# Autodesk Inventor assembly: TS_V1_Fallmagazin_gesamt
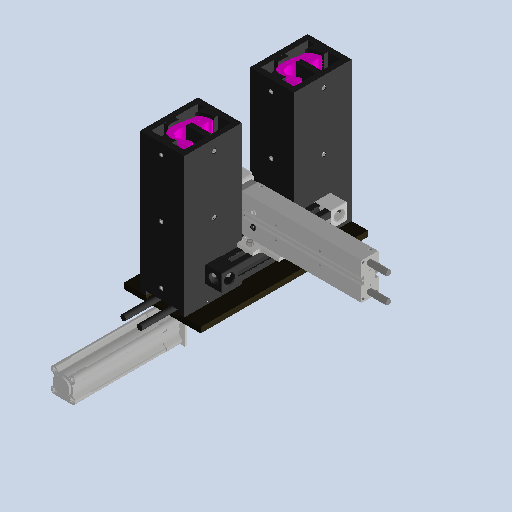
[picture p0: Inventor's stored thumbnail of the model, 512x512]
Saved by Autodesk Inventor 2025.2 (Build 292293000, 293)
## iProperties
Created: 2025-06-10
Part Number: TS_V1_Fallmagazin_gesamt
Document SubType Name: Assembly
Designer: tino
Author: tino
## Documents named in this file (30)
- C:\Users\tino\Documents_VM\Konst_CAD\CAD-Paspa\Useless Box\Eigene Bauteile\Fallmagazin\TS_V1_Fallmagazin_gesamt.iam
- C:\Users\tino\Documents_VM\Konst_CAD\CAD-Paspa\Useless Box\Eigene Bauteile\Fallmagazin\TS_V1_Fallmagazin_Boden_int.ipt
- C:\Users\tino\Documents_VM\Konst_CAD\CAD-Paspa\Useless Box\Eigene Bauteile\Fallmagazin\TS_V1_Fallmagazin_Wandung_int.ipt
- C:\Users\tino\Documents_VM\Konst_CAD\CAD-Paspa\Useless Box\Eigene Bauteile\Fallmagazin\TS_V1_Fallmagazin_Leitbleche_vorne_int.ipt
- C:\Users\tino\Documents_VM\Konst_CAD\CAD-Paspa\Useless Box\_Useless_Box\Finger.ipt
- C:\Users\tino\Documents_VM\Konst_CAD\CAD-Paspa\Useless Box\Eigene Bauteile\Fallmagazin\TS_V1_Fallmagazin_Schieber.iam
- C:\Users\tino\Documents_VM\Konst_CAD\CAD-Paspa\Useless Box\Kaufteile\Festo_Normzylinder_100\1376426 DSBC-32-100-PPVA-N3---(0).iam
- C:\Users\tino\Documents_VM\Konst_CAD\CAD-Paspa\Useless Box\Standart Bauteile\ISO 4762 - M4 x 12ISO.ipt
- C:\Users\tino\Documents_VM\Konst_CAD\CAD-Paspa\Useless Box\Standart Bauteile\ISO 4762 - M4 x 16ISO.ipt
- C:\Users\tino\Documents_VM\Konst_CAD\CAD-Paspa\Useless Box\Eigene Bauteile\Fallmagazin\TS_V1_Fallmagazin_Zylinderanbindung_int.ipt
- C:\Users\tino\Documents_VM\Konst_CAD\CAD-Paspa\Useless Box\Eigene Bauteile\Fallmagazin\TS_V1_Fallmagazin_Stopper_int.ipt
- C:\Users\tino\Documents_VM\Konst_CAD\CAD-Paspa\Useless Box\Eigene Bauteile\Fallmagazin\TS_V1_Fallmagazin_Zylinderhalter_int.ipt
- C:\Users\tino\Documents_VM\Konst_CAD\CAD-Paspa\Useless Box\Standart Bauteile\ISO 4762 - M5 x 8ISO.ipt
- C:\Users\tino\Documents_VM\Konst_CAD\CAD-Paspa\Useless Box\Standart Bauteile\ISO 4762 - M5 x 20ISO.ipt
- C:\Users\tino\Documents_VM\Konst_CAD\CAD-Paspa\Useless Box\Standart Bauteile\DIN EN ISO 2338 - 4 m6 x 10.ipt
- C:\Users\tino\Documents_VM\Konst_CAD\CAD-Paspa\Useless Box\Standart Bauteile\DIN 7991 - M5x12.ipt
- C:\Users\tino\Documents_VM\Konst_CAD\CAD-Paspa\Useless Box\Eigene Bauteile\Fallmagazin\TS_V1_Fallmagazin_Schieberanbindung_int.ipt
- C:\Users\tino\Documents_VM\Konst_CAD\CAD-Paspa\Useless Box\Eigene Bauteile\Fallmagazin\TS_V1_Fallmagazin_Verbindungsstange_int.ipt
- C:\Users\tino\Documents_VM\Konst_CAD\CAD-Paspa\Useless Box\Kaufteile\Festo_Fuehrungszylinder150_DFM_16\529120 DFM-16-150-B-P-A-KF---(0).iam
- C:\Users\tino\Documents_VM\Konst_CAD\CAD-Paspa\Useless Box\Kaufteile\DHRS-32-A - Kopie\AIS2024\1310164 DHRS-32-A---(0).iam
- C:\Users\tino\Documents_VM\Konst_CAD\CAD-Paspa\Useless Box\Eigene Bauteile\TS_Adapter_Greifer_int.ipt
- C:\Users\tino\Documents_VM\Konst_CAD\CAD-Paspa\Useless Box\Standart Bauteile\ISO 4762 - M4 x 10ISO.ipt
- C:\Users\tino\Documents_VM\Konst_CAD\CAD-Paspa\Useless Box\Eigene Bauteile\TS_Halterung_Fuehrungszylinder_int.ipt
- C:\Users\tino\Documents_VM\Konst_CAD\CAD-Paspa\Useless Box\Kaufteile\Rexroth_Profil+Winkel_30x30\Rexroth_30x30_Wuerfel\Rexroth_30x30_Wuerfel\Rexroth_30x30_Wuerfel.ipt
- C:\Users\tino\Documents_VM\Konst_CAD\CAD-Paspa\Useless Box\Kaufteile\Rexroth_Profil+Winkel_30x30\Rexroth_30x30_200_ext\Rexroth_30x30_200_ext\Rexroth_30x30_200_ext.ipt
- C:\Users\tino\Documents_VM\Konst_CAD\CAD-Paspa\Useless Box\Standart Bauteile\DIN 7991 - M8x16.ipt
- C:\Users\tino\Documents_VM\Konst_CAD\CAD-Paspa\Useless Box\Standart Bauteile\DIN 934 - M5 x 0,8.ipt
- C:\Users\tino\Documents_VM\Konst_CAD\CAD-Paspa\Useless Box\Standart Bauteile\ISO 4762 - M6 x 12ISO.ipt
- C:\Users\tino\Documents_VM\Konst_CAD\CAD-Paspa\Useless Box\Kaufteile\Rexroth_Hammermuttern\Rexroth_Hammermutter_8_M6\Rexroth_Hammermutter_8_M6\Rexroth_Hammermutter_8_M6.ipt
- C:\Users\tino\Documents_VM\Konst_CAD\CAD-Paspa\Useless Box\Standart Bauteile\DIN 913 - M5 x 6.ipt
## Components (190 placed, 29 different names)
1. TS_V1_Fallmagazin_Boden_int:1 — Passend:16, Passend:17, Passend:21, Passend:23, Passend:25, Passend:26, Passend:30, Passend:43, Passend:44, Passend:45, Passend:46, Fluchtend:18, Passend:84, Passend:85, Passend:86, Passend:87, Passend:94, Passend:96, Passend:97, Fluchtend:19, Fluchtend:20, Passend:121
2. TS_V1_Fallmagazin_Wandung_int:2 — Passend:7, Passend:8, Fluchtend:4, Winkel:1, Winkel:2, Passend:16, Passend:17, Passend:35, Passend:36, Passend:37, Passend:38, Passend:39, Passend:40, Passend:41, Passend:42, Winkel:3, Passend:130
3. TS_V1_Fallmagazin_Leitbleche_vorne_int:1 — Passend:7, Passend:8, Fluchtend:4, Tangential:2, Tangential:5, Fluchtend:12
4. TS_V1_Fallmagazin_Schieber:1 [sub-assembly] — Passend:21, Passend:25, Passend:26, Passend:53, Passend:61, Passend:62, Passend:63, Passend:64, Passend:106, Tangential:6
5. TS_V1_Fallmagazin_Schieber:2 [sub-assembly] — Passend:23, Passend:30, Passend:65, Passend:66, Passend:67, Passend:101, Passend:103, Passend:107
6. 1376426 DSBC-32-100-PPVA-N3---(0):1 [sub-assembly] — Fluchtend:18, Passend:68, Passend:69, Passend:92, Passend:93, Passend:99
7. TS_V1_Fallmagazin_Wandung_int:3 — Passend:45, Passend:46, Passend:47, Fluchtend:14, Passend:48, Passend:132, Passend:137, Passend:138
8. TS_V1_Fallmagazin_Leitbleche_vorne_int:2 — Passend:47, Fluchtend:14, Passend:48
9. TS_V1_Fallmagazin_Zylinderanbindung_int:1 — Passend:53, Passend:99, Winkel:4, Passend:104, Passend:108, Passend:110, Passend:144
10. TS_V1_Fallmagazin_Stopper_int:1 — Passend:61, Passend:62, Winkel:3
11. TS_V1_Fallmagazin_Stopper_int:2 — Passend:63, Passend:64
12. TS_V1_Fallmagazin_Stopper_int:3 — Passend:65, Fluchtend:16, Passend:67
13. TS_V1_Fallmagazin_Stopper_int:4 — Passend:66, Fluchtend:16
14. TS_V1_Fallmagazin_Zylinderhalter_int:1 — Passend:68, Passend:69, Passend:71, Passend:72, Passend:90, Passend:91, Passend:93, Passend:95, Passend:97
15. DIN 7991 M5x12:1 — Passend:106, Tangential:6, Passend:108
16. DIN 7991 M5x12:2 — Passend:101, Passend:107, Passend:109
17. TS_V1_Fallmagazin_Schieberanbindung_int:1 — Winkel:4, Passend:103, Passend:105, Passend:109, Passend:142
18. TS_V1_Fallmagazin_Verbindungsstange_int:1 — Passend:104, Passend:105, Winkel:5, Passend:110, Passend:141, Passend:143
19. 529120 DFM-16-150-B-P-A-KF---(0):1 [sub-assembly] — Fluchtend:19, Winkel:6, Fluchtend:21, Passend:116, Passend:117, Passend:120, Passend:121, Passend:122, Passend:123, Passend:124, Winkel:7, Winkel:8
20. 1310164 DHRS-32-A---(0):1 [sub-assembly] — Fluchtend:20, Fluchtend:21, Passend:113, Passend:118, Passend:119, Passend:153
21. TS_Adapter_Greifer_int:1 — Passend:113, Passend:114, Passend:115, Passend:118, Passend:119, Passend:120, Passend:153, Passend:154, Fluchtend:26
22. TS_Halterung_Fuehrungszylinder_int:1 — Passend:122, Passend:123, Passend:124, Passend:135, Passend:145, Passend:146, Passend:147, Passend:148, Passend:150, Passend:151, Passend:152
23. Rexroth_30x30_Wuerfel:1 — Passend:130, Passend:134, Fluchtend:24, Fluchtend:25, Passend:136, Tangential:7, Passend:139, Tangential:9
24. Rexroth_30x30_Wuerfel:2 — Passend:132, Passend:133, Fluchtend:22, Fluchtend:23, Passend:137, Tangential:8, Passend:140, Tangential:10
25. Rexroth_30x30_170_ext:1 — Passend:133, Fluchtend:22, Fluchtend:23, Passend:134, Fluchtend:24, Fluchtend:25, Passend:135, Tangential:11, Tangential:12
26. DIN 7991 M8x16:3 — Passend:136, Tangential:7
27. DIN 7991 M8x16:4 — Passend:138, Tangential:8
28. DIN 7991 M8x16:5 — Passend:139, Tangential:9
29. DIN 7991 M8x16:6 — Passend:140, Tangential:10
30. DIN 934 - M5 x 0,8:1 — Passend:141, Passend:142
31. DIN 934 - M5 x 0,8:2 — Passend:143, Passend:144
32. ISO 4762 - M6 x 12ISO:1 — Passend:147, Passend:148, Passend:149
33. Rexroth_Hammermutter_8_M6:1 — Winkel:7, Tangential:11, Passend:149
34. Rexroth_Hammermutter_8_M6:2 — Winkel:8, Tangential:12, Passend:150
35. ISO 4762 - M6 x 12ISO:2 — Passend:151, Passend:152
36. DIN 913 - M5 x 6:1 — Passend:154, Fluchtend:26
37. Finger:1 — Winkel:1, Tangential:2, Tangential:5, Winkel:2, Fluchtend:12
38. Finger:2
39. Finger:3
40. Finger:4
41. Finger:5
42. Finger:6
43. Finger:7
44. Finger:8
45. Finger:9
46. Finger:10
47. Finger:11
48. Finger:12
49. Finger:13
50. Finger:14
51. Finger:15
52. Finger:16
53. Finger:17
54. Finger:18
55. Finger:19
56. Finger:20
57. Finger:21
58. Finger:22
59. Finger:23
60. Finger:24
61. Finger:25
62. Finger:26
63. Finger:27
64. Finger:28
65. Finger:29
66. Finger:30
67. Finger:31
68. Finger:32
69. Finger:33
70. Finger:34
71. Finger:35
72. Finger:36
73. Finger:37
74. Finger:38
75. Finger:39
76. Finger:40
77. Finger:41
78. Finger:42
79. Finger:43
80. Finger:44
81. Finger:45
82. Finger:46
83. Finger:47
84. Finger:48
85. Finger:49
86. Finger:50
87. Finger:51
88. Finger:52
89. Finger:53
90. Finger:54
91. Finger:55
92. Finger:56
93. Finger:57
94. Finger:58
95. Finger:59
96. Finger:60
97. Finger:61
98. Finger:62
99. Finger:63
100. Finger:64
101. Finger:65
102. Finger:66
103. Finger:67
104. Finger:68
105. Finger:69
106. Finger:70
107. Finger:71
108. Finger:72
109. Finger:73
110. Finger:74
111. Finger:75
112. Finger:76
113. Finger:77
114. Finger:78
115. Finger:79
116. Finger:80
117. Finger:81
118. Finger:82
119. Finger:83
120. Finger:84
121. Finger:85
122. Finger:86
123. Finger:87
124. Finger:88
125. Finger:89
126. Finger:90
127. Finger:91
128. Finger:92
129. Finger:93
130. Finger:94
131. Finger:95
132. Finger:96
133. Finger:97
134. Finger:98
135. ISO 4762 M5 x 8:1 — Passend:71, Passend:72, Passend:96
136. ISO 4762 M5 x 8:2
137. ISO 4762 M5 x 8:3 — Passend:94
138. ISO 4762 M5 x 8:4
139. ISO 4762 M5 x 20:1 — Passend:92, Passend:95
140. ISO 4762 M5 x 20:2 — Passend:91
141. ISO 4762 M5 x 20:3 — Passend:90
142. ISO 4762 M5 x 20:4
143. ISO 4762 M4 x 10:1 — Passend:114, Passend:115, Passend:116
144. ISO 4762 M4 x 10:2 — Passend:117
145. ISO 4762 M4 x 10:3
146. ISO 4762 M4 x 10:4
147. DIN EN ISO 2338 4 m6 x 10:1 — Passend:84, Passend:85
148. DIN EN ISO 2338 4 m6 x 10:2 — Passend:86, Passend:87
149. DIN EN ISO 2338 4 m6 x 10:3
150. DIN EN ISO 2338 4 m6 x 10:4
151. ISO 4762 M4 x 10:5 — Passend:145, Passend:146
152. ISO 4762 M4 x 10:6
153. ISO 4762 M4 x 10:7
154. ISO 4762 M4 x 10:8
155. ISO 4762 M4 x 12:1 — Passend:35, Passend:36
156. ISO 4762 M4 x 12:2
157. ISO 4762 M4 x 12:3
158. ISO 4762 M4 x 12:4 — Passend:37, Passend:38
159. ISO 4762 M4 x 12:5
160. ISO 4762 M4 x 12:6
161. ISO 4762 M4 x 12:7 — Passend:39, Passend:40
162. ISO 4762 M4 x 12:8
163. ISO 4762 M4 x 12:9
164. ISO 4762 M4 x 12:10 — Passend:41, Passend:42
165. ISO 4762 M4 x 12:11
166. ISO 4762 M4 x 12:12
167. ISO 4762 M4 x 16:1 — Passend:43, Passend:44
168. ISO 4762 M4 x 16:2
169. ISO 4762 M4 x 16:3
170. ISO 4762 M4 x 16:4
171. ISO 4762 M4 x 16:5
172. ISO 4762 M4 x 16:6
173. ISO 4762 M4 x 12:13
174. ISO 4762 M4 x 12:14
175. ISO 4762 M4 x 12:15
176. ISO 4762 M4 x 12:16
177. ISO 4762 M4 x 12:17
178. ISO 4762 M4 x 12:18
179. ISO 4762 M4 x 12:19
180. ISO 4762 M4 x 12:20
181. ISO 4762 M4 x 12:21
182. ISO 4762 M4 x 12:22
183. ISO 4762 M4 x 12:23
184. ISO 4762 M4 x 12:24
185. ISO 4762 M4 x 16:7
186. ISO 4762 M4 x 16:8
187. ISO 4762 M4 x 16:9
188. ISO 4762 M4 x 16:10
189. ISO 4762 M4 x 16:11
190. ISO 4762 M4 x 16:12
## Component patterns: (2 elements), (98 elements, first: Finger:1), (4 elements, first: ISO 4762 M5 x 8:1), (4 elements, first: ISO 4762 M5 x 20:1), (4 elements, first: ISO 4762 M4 x 10:1), (2 elements, first: DIN EN ISO 2338 4 m6 x 10:1 + DIN EN ISO 2338 4 m6 x 10:2), (4 elements, first: ISO 4762 M4 x 10:5), (3 elements, first: ISO 4762 M4 x 12:1), (3 elements, first: ISO 4762 M4 x 12:4), (3 elements, first: ISO 4762 M4 x 12:7), (3 elements, first: ISO 4762 M4 x 12:10), (6 elements, first: ISO 4762 M4 x 16:1), Komponentenanordnung 2:2 (3 elements), Komponentenanordnung 3:2 (3 elements), Komponentenanordnung 4:2 (3 elements), Komponentenanordnung 5:2 (3 elements), Komponentenanordnung 6:2 (6 elements)
## Relationships (123: Mate 93, Flush 13, Tangent 9, Angle 8)
- Passend:7 [Mate]: TS_V1_Fallmagazin_Wandung_int:2 ↔ TS_V1_Fallmagazin_Leitbleche_vorne_int:1
- Passend:8 [Mate]: TS_V1_Fallmagazin_Wandung_int:2 ↔ TS_V1_Fallmagazin_Leitbleche_vorne_int:1
- Fluchtend:4 [Flush]: TS_V1_Fallmagazin_Wandung_int:2 ↔ TS_V1_Fallmagazin_Leitbleche_vorne_int:1
- Winkel:1 [Angle] (0 deg): TS_V1_Fallmagazin_Wandung_int:2 ↔ Finger:1
- Tangential:2: TS_V1_Fallmagazin_Leitbleche_vorne_int:1 ↔ Finger:1
- Tangential:5: TS_V1_Fallmagazin_Leitbleche_vorne_int:1 ↔ Finger:1
- Winkel:2 [Angle] (0 deg): TS_V1_Fallmagazin_Wandung_int:2 ↔ Finger:1
- Passend:16 [Mate]: TS_V1_Fallmagazin_Boden_int:1 ↔ TS_V1_Fallmagazin_Wandung_int:2
- Passend:17 [Mate]: TS_V1_Fallmagazin_Boden_int:1 ↔ TS_V1_Fallmagazin_Wandung_int:2
- Passend:21 [Mate]: TS_V1_Fallmagazin_Boden_int:1 ↔ TS_V1_Fallmagazin_Schieber:1
- Passend:23 [Mate]: TS_V1_Fallmagazin_Boden_int:1 ↔ TS_V1_Fallmagazin_Schieber:2
- Passend:25 [Mate]: TS_V1_Fallmagazin_Boden_int:1 ↔ TS_V1_Fallmagazin_Schieber:1
- Passend:26 [Mate]: TS_V1_Fallmagazin_Boden_int:1 ↔ TS_V1_Fallmagazin_Schieber:1
- Passend:30 [Mate]: TS_V1_Fallmagazin_Boden_int:1 ↔ TS_V1_Fallmagazin_Schieber:2
- Passend:35 [Mate]: TS_V1_Fallmagazin_Wandung_int:2 ↔ ISO 4762 M4 x 12:1
- Passend:36 [Mate]: TS_V1_Fallmagazin_Wandung_int:2 ↔ ISO 4762 M4 x 12:1
- Passend:37 [Mate]: TS_V1_Fallmagazin_Wandung_int:2 ↔ ISO 4762 M4 x 12:4
- Passend:38 [Mate]: TS_V1_Fallmagazin_Wandung_int:2 ↔ ISO 4762 M4 x 12:4
- Passend:39 [Mate]: TS_V1_Fallmagazin_Wandung_int:2 ↔ ISO 4762 M4 x 12:7
- Passend:40 [Mate]: TS_V1_Fallmagazin_Wandung_int:2 ↔ ISO 4762 M4 x 12:7
- Passend:41 [Mate]: TS_V1_Fallmagazin_Wandung_int:2 ↔ ISO 4762 M4 x 12:10
- Passend:42 [Mate]: TS_V1_Fallmagazin_Wandung_int:2 ↔ ISO 4762 M4 x 12:10
- Passend:43 [Mate]: TS_V1_Fallmagazin_Boden_int:1 ↔ ISO 4762 M4 x 16:1
- Passend:44 [Mate]: TS_V1_Fallmagazin_Boden_int:1 ↔ ISO 4762 M4 x 16:1
- Fluchtend:12 [Flush]: TS_V1_Fallmagazin_Leitbleche_vorne_int:1 ↔ Finger:1
- Passend:45 [Mate]: TS_V1_Fallmagazin_Boden_int:1 ↔ TS_V1_Fallmagazin_Wandung_int:3
- Passend:46 [Mate]: TS_V1_Fallmagazin_Boden_int:1 ↔ TS_V1_Fallmagazin_Wandung_int:3
- Passend:47 [Mate]: TS_V1_Fallmagazin_Wandung_int:3 ↔ TS_V1_Fallmagazin_Leitbleche_vorne_int:2
- Fluchtend:14 [Flush]: TS_V1_Fallmagazin_Wandung_int:3 ↔ TS_V1_Fallmagazin_Leitbleche_vorne_int:2
- Passend:48 [Mate]: TS_V1_Fallmagazin_Wandung_int:3 ↔ TS_V1_Fallmagazin_Leitbleche_vorne_int:2
- Passend:53 [Mate]: TS_V1_Fallmagazin_Schieber:1 ↔ TS_V1_Fallmagazin_Zylinderanbindung_int:1
- Passend:61 [Mate]: TS_V1_Fallmagazin_Schieber:1 ↔ TS_V1_Fallmagazin_Stopper_int:1
- Passend:62 [Mate]: TS_V1_Fallmagazin_Schieber:1 ↔ TS_V1_Fallmagazin_Stopper_int:1
- Passend:63 [Mate]: TS_V1_Fallmagazin_Schieber:1 ↔ TS_V1_Fallmagazin_Stopper_int:2
- Passend:64 [Mate]: TS_V1_Fallmagazin_Schieber:1 ↔ TS_V1_Fallmagazin_Stopper_int:2
- Passend:65 [Mate]: TS_V1_Fallmagazin_Schieber:2 ↔ TS_V1_Fallmagazin_Stopper_int:3
- Passend:66 [Mate]: TS_V1_Fallmagazin_Schieber:2 ↔ TS_V1_Fallmagazin_Stopper_int:4
- Fluchtend:16 [Flush]: TS_V1_Fallmagazin_Stopper_int:3 ↔ TS_V1_Fallmagazin_Stopper_int:4
- Passend:67 [Mate]: TS_V1_Fallmagazin_Schieber:2 ↔ TS_V1_Fallmagazin_Stopper_int:3
- Fluchtend:18 [Flush]: TS_V1_Fallmagazin_Boden_int:1 ↔ 1376426 DSBC-32-100-PPVA-N3---(0):1
- Passend:68 [Mate]: 1376426 DSBC-32-100-PPVA-N3---(0):1 ↔ TS_V1_Fallmagazin_Zylinderhalter_int:1
- Passend:69 [Mate]: 1376426 DSBC-32-100-PPVA-N3---(0):1 ↔ TS_V1_Fallmagazin_Zylinderhalter_int:1
- Passend:71 [Mate]: TS_V1_Fallmagazin_Zylinderhalter_int:1 ↔ ISO 4762 M5 x 8:1
- Passend:72 [Mate]: TS_V1_Fallmagazin_Zylinderhalter_int:1 ↔ ISO 4762 M5 x 8:1
- Passend:84 [Mate]: TS_V1_Fallmagazin_Boden_int:1 ↔ DIN EN ISO 2338 4 m6 x 10:1
- Passend:85 [Mate] (0.5 mm): TS_V1_Fallmagazin_Boden_int:1 ↔ DIN EN ISO 2338 4 m6 x 10:1
- Passend:86 [Mate]: TS_V1_Fallmagazin_Boden_int:1 ↔ DIN EN ISO 2338 4 m6 x 10:2
- Passend:87 [Mate] (1 mm): TS_V1_Fallmagazin_Boden_int:1 ↔ DIN EN ISO 2338 4 m6 x 10:2
- Winkel:3 [Angle] (0 deg): TS_V1_Fallmagazin_Wandung_int:2 ↔ TS_V1_Fallmagazin_Stopper_int:1
- Passend:90 [Mate]: TS_V1_Fallmagazin_Zylinderhalter_int:1 ↔ ISO 4762 M5 x 20:3
- Passend:91 [Mate]: TS_V1_Fallmagazin_Zylinderhalter_int:1 ↔ ISO 4762 M5 x 20:2
- Passend:92 [Mate]: 1376426 DSBC-32-100-PPVA-N3---(0):1 ↔ ISO 4762 M5 x 20:1
- Passend:93 [Mate]: 1376426 DSBC-32-100-PPVA-N3---(0):1 ↔ TS_V1_Fallmagazin_Zylinderhalter_int:1
- Passend:94 [Mate]: TS_V1_Fallmagazin_Boden_int:1 ↔ ISO 4762 M5 x 8:3
- Passend:95 [Mate]: TS_V1_Fallmagazin_Zylinderhalter_int:1 ↔ ISO 4762 M5 x 20:1
- Passend:96 [Mate]: TS_V1_Fallmagazin_Boden_int:1 ↔ ISO 4762 M5 x 8:1
- Passend:97 [Mate]: TS_V1_Fallmagazin_Boden_int:1 ↔ TS_V1_Fallmagazin_Zylinderhalter_int:1
- Passend:99 [Mate]: 1376426 DSBC-32-100-PPVA-N3---(0):1 ↔ TS_V1_Fallmagazin_Zylinderanbindung_int:1
- Passend:101 [Mate]: TS_V1_Fallmagazin_Schieber:2 ↔ DIN 7991 M5x12:2
- Winkel:4 [Angle] (180 deg): TS_V1_Fallmagazin_Zylinderanbindung_int:1 ↔ TS_V1_Fallmagazin_Schieberanbindung_int:1
- Passend:103 [Mate]: TS_V1_Fallmagazin_Schieber:2 ↔ TS_V1_Fallmagazin_Schieberanbindung_int:1
- Passend:104 [Mate]: TS_V1_Fallmagazin_Zylinderanbindung_int:1 ↔ TS_V1_Fallmagazin_Verbindungsstange_int:1
- Passend:105 [Mate] (-10 mm): TS_V1_Fallmagazin_Schieberanbindung_int:1 ↔ TS_V1_Fallmagazin_Verbindungsstange_int:1
- Winkel:5 [Angle] (0 deg): TS_V1_Fallmagazin_Verbindungsstange_int:1
- Passend:106 [Mate]: TS_V1_Fallmagazin_Schieber:1 ↔ DIN 7991 M5x12:1
- Tangential:6: TS_V1_Fallmagazin_Schieber:1 ↔ DIN 7991 M5x12:1
- Passend:107 [Mate]: TS_V1_Fallmagazin_Schieber:2 ↔ DIN 7991 M5x12:2
- Passend:108 [Mate]: TS_V1_Fallmagazin_Zylinderanbindung_int:1 ↔ DIN 7991 M5x12:1
- Passend:109 [Mate]: DIN 7991 M5x12:2 ↔ TS_V1_Fallmagazin_Schieberanbindung_int:1
- Passend:110 [Mate] (-10 mm): TS_V1_Fallmagazin_Zylinderanbindung_int:1 ↔ TS_V1_Fallmagazin_Verbindungsstange_int:1
- Fluchtend:19 [Flush] (22.694 mm): TS_V1_Fallmagazin_Boden_int:1 ↔ 529120 DFM-16-150-B-P-A-KF---(0):1
- Winkel:6 [Angle] (0 deg): 529120 DFM-16-150-B-P-A-KF---(0):1
- Fluchtend:20 [Flush] (-135 mm): TS_V1_Fallmagazin_Boden_int:1 ↔ 1310164 DHRS-32-A---(0):1
- Fluchtend:21 [Flush]: 529120 DFM-16-150-B-P-A-KF---(0):1 ↔ 1310164 DHRS-32-A---(0):1
- Passend:113 [Mate]: 1310164 DHRS-32-A---(0):1 ↔ TS_Adapter_Greifer_int:1
- Passend:114 [Mate]: TS_Adapter_Greifer_int:1 ↔ ISO 4762 M4 x 10:1
- Passend:115 [Mate]: TS_Adapter_Greifer_int:1 ↔ ISO 4762 M4 x 10:1
- Passend:116 [Mate]: 529120 DFM-16-150-B-P-A-KF---(0):1 ↔ ISO 4762 M4 x 10:1
- Passend:117 [Mate]: 529120 DFM-16-150-B-P-A-KF---(0):1 ↔ ISO 4762 M4 x 10:2
- Passend:118 [Mate]: 1310164 DHRS-32-A---(0):1 ↔ TS_Adapter_Greifer_int:1
- Passend:119 [Mate]: 1310164 DHRS-32-A---(0):1 ↔ TS_Adapter_Greifer_int:1
- Passend:120 [Mate]: 529120 DFM-16-150-B-P-A-KF---(0):1 ↔ TS_Adapter_Greifer_int:1
- Passend:121 [Mate] (30.575 mm): TS_V1_Fallmagazin_Boden_int:1 ↔ 529120 DFM-16-150-B-P-A-KF---(0):1
- Passend:122 [Mate]: 529120 DFM-16-150-B-P-A-KF---(0):1 ↔ TS_Halterung_Fuehrungszylinder_int:1
- Passend:123 [Mate]: 529120 DFM-16-150-B-P-A-KF---(0):1 ↔ TS_Halterung_Fuehrungszylinder_int:1
- Passend:124 [Mate]: 529120 DFM-16-150-B-P-A-KF---(0):1 ↔ TS_Halterung_Fuehrungszylinder_int:1
- Passend:130 [Mate]: TS_V1_Fallmagazin_Wandung_int:2 ↔ Rexroth_30x30_Wuerfel:1
- Passend:132 [Mate]: TS_V1_Fallmagazin_Wandung_int:3 ↔ Rexroth_30x30_Wuerfel:2
- Passend:133 [Mate]: Rexroth_30x30_Wuerfel:2 ↔ Rexroth_30x30_170_ext:1
- Fluchtend:22 [Flush]: Rexroth_30x30_Wuerfel:2 ↔ Rexroth_30x30_170_ext:1
- Fluchtend:23 [Flush]: Rexroth_30x30_Wuerfel:2 ↔ Rexroth_30x30_170_ext:1
- Passend:134 [Mate]: Rexroth_30x30_Wuerfel:1 ↔ Rexroth_30x30_170_ext:1
- Fluchtend:24 [Flush]: Rexroth_30x30_Wuerfel:1 ↔ Rexroth_30x30_170_ext:1
- Fluchtend:25 [Flush]: Rexroth_30x30_Wuerfel:1 ↔ Rexroth_30x30_170_ext:1
- Passend:135 [Mate]: TS_Halterung_Fuehrungszylinder_int:1 ↔ Rexroth_30x30_170_ext:1
- Passend:136 [Mate]: Rexroth_30x30_Wuerfel:1 ↔ DIN 7991 M8x16:3
- Tangential:7: Rexroth_30x30_Wuerfel:1 ↔ DIN 7991 M8x16:3
- Passend:137 [Mate]: TS_V1_Fallmagazin_Wandung_int:3 ↔ Rexroth_30x30_Wuerfel:2
- Passend:138 [Mate]: TS_V1_Fallmagazin_Wandung_int:3 ↔ DIN 7991 M8x16:4
- Tangential:8: Rexroth_30x30_Wuerfel:2 ↔ DIN 7991 M8x16:4
- Passend:139 [Mate]: Rexroth_30x30_Wuerfel:1 ↔ DIN 7991 M8x16:5
- Tangential:9: Rexroth_30x30_Wuerfel:1 ↔ DIN 7991 M8x16:5
- Passend:140 [Mate]: Rexroth_30x30_Wuerfel:2 ↔ DIN 7991 M8x16:6
- Tangential:10: Rexroth_30x30_Wuerfel:2 ↔ DIN 7991 M8x16:6
- Passend:141 [Mate]: TS_V1_Fallmagazin_Verbindungsstange_int:1 ↔ DIN 934 - M5 x 0,8:1
- Passend:142 [Mate]: TS_V1_Fallmagazin_Schieberanbindung_int:1 ↔ DIN 934 - M5 x 0,8:1
- Passend:143 [Mate]: TS_V1_Fallmagazin_Verbindungsstange_int:1 ↔ DIN 934 - M5 x 0,8:2
- Passend:144 [Mate]: TS_V1_Fallmagazin_Zylinderanbindung_int:1 ↔ DIN 934 - M5 x 0,8:2
- Passend:145 [Mate]: TS_Halterung_Fuehrungszylinder_int:1 ↔ ISO 4762 M4 x 10:5
- Passend:146 [Mate]: TS_Halterung_Fuehrungszylinder_int:1 ↔ ISO 4762 M4 x 10:5
- Passend:147 [Mate]: TS_Halterung_Fuehrungszylinder_int:1 ↔ ISO 4762 - M6 x 12ISO:1
- Passend:148 [Mate]: TS_Halterung_Fuehrungszylinder_int:1 ↔ ISO 4762 - M6 x 12ISO:1
- Winkel:7 [Angle] (180 deg): 529120 DFM-16-150-B-P-A-KF---(0):1 ↔ Rexroth_Hammermutter_8_M6:1
- Tangential:11: Rexroth_30x30_170_ext:1 ↔ Rexroth_Hammermutter_8_M6:1
- Passend:149 [Mate]: ISO 4762 - M6 x 12ISO:1 ↔ Rexroth_Hammermutter_8_M6:1
- Winkel:8 [Angle] (0 deg): 529120 DFM-16-150-B-P-A-KF---(0):1 ↔ Rexroth_Hammermutter_8_M6:2
- Tangential:12: Rexroth_30x30_170_ext:1 ↔ Rexroth_Hammermutter_8_M6:2
- Passend:150 [Mate]: TS_Halterung_Fuehrungszylinder_int:1 ↔ Rexroth_Hammermutter_8_M6:2
- Passend:151 [Mate]: TS_Halterung_Fuehrungszylinder_int:1 ↔ ISO 4762 - M6 x 12ISO:2
- Passend:152 [Mate]: TS_Halterung_Fuehrungszylinder_int:1 ↔ ISO 4762 - M6 x 12ISO:2
- Passend:153 [Mate]: 1310164 DHRS-32-A---(0):1 ↔ TS_Adapter_Greifer_int:1
- Passend:154 [Mate]: TS_Adapter_Greifer_int:1 ↔ DIN 913 - M5 x 6:1
- Fluchtend:26 [Flush]: TS_Adapter_Greifer_int:1 ↔ DIN 913 - M5 x 6:1
## Named parameters: Magazin_Hoehe = 255 mm, Abstand_Schrauben_vert = 105 mm, Abstand_Rand = 45 mm, Anbindung_Zylinder = 16.4 mm
